# Autodesk Inventor assembly: Full Energy Chain Tensioner
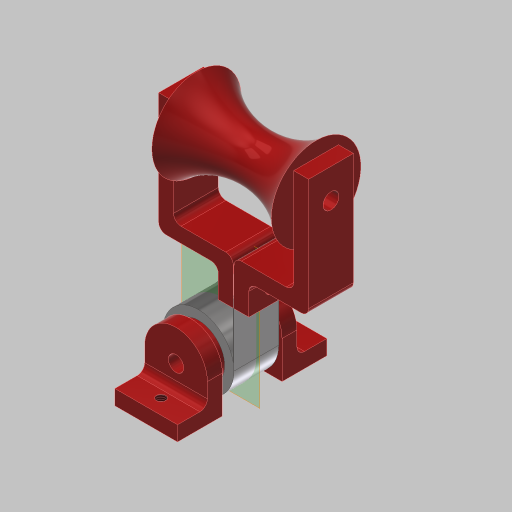
[picture p0: Inventor's stored thumbnail of the model, 512x512]
Saved by Autodesk Inventor 2023.5 (Build 275446000, 446)
## iProperties
Created: 2025-02-13
Part Number: Full Energy Chain Tensioner
Document SubType Name: Assembly
Designer: slick
Author: slick
## Documents named in this file (5)
- C:\Users\slick\OneDrive\Desktop\2025-ReefScape---CAD\Elevator\EL2\Full Energy Chain Tensioner.iam
- C:\Users\slick\OneDrive\Desktop\2025-ReefScape---CAD\Elevator\EL2\Energy Chain Tensioner piece.iam
- C:\Users\slick\OneDrive\Desktop\2025-ReefScape---CAD\Elevator\EL2\EL2-030.ipt
- C:\Users\slick\OneDrive\Desktop\2025-ReefScape---CAD\Elevator\EL2\EL2-029.ipt
- C:\Users\slick\OneDrive\Desktop\2025-ReefScape---CAD\COMMON PARTS\BEARINGS\Ball Bearing 1_4x11_16x5_16 Sealed 1602DC 1602-2RS.ipt
## Components (6 placed, 4 different names)
1. Energy Chain Tensioner piece:1 [sub-assembly] — Mate:1, Mate:2, Mate:3, Angle:1
2. EL2-030:1 — Flush:1, Flush:2, Mate:2, Angle:1, Mate:7
3. EL2-030:2 — Flush:1, Flush:2, Mate:1, Mate:3, Mate:6
4. EL2-029:1 — Mate:4, Mate:5, Flush:3, Flush:4
5. Ball Bearing 1_4x11_16x5_16 Sealed 1602DC 1602-2RS:1 — Mate:5, Flush:3, Mate:7
6. Ball Bearing 1_4x11_16x5_16 Sealed 1602DC 1602-2RS:2 — Mate:4, Flush:4, Mate:6
## Relationships (12: Mate 7, Flush 4, Angle 1)
- Flush:1: EL2-030:1 ↔ EL2-030:2
- Flush:2: EL2-030:1 ↔ EL2-030:2
- Mate:1: Energy Chain Tensioner piece:1 ↔ EL2-030:2
- Mate:2: Energy Chain Tensioner piece:1 ↔ EL2-030:1
- Mate:3: Energy Chain Tensioner piece:1 ↔ EL2-030:2
- Angle:1 (0 deg): Energy Chain Tensioner piece:1 ↔ EL2-030:1
- Mate:4: EL2-029:1 ↔ Ball Bearing 1_4x11_16x5_16 Sealed 1602DC 1602-2RS:2
- Mate:5: EL2-029:1 ↔ Ball Bearing 1_4x11_16x5_16 Sealed 1602DC 1602-2RS:1
- Flush:3: EL2-029:1 ↔ Ball Bearing 1_4x11_16x5_16 Sealed 1602DC 1602-2RS:1
- Flush:4: EL2-029:1 ↔ Ball Bearing 1_4x11_16x5_16 Sealed 1602DC 1602-2RS:2
- Mate:6: EL2-030:2 ↔ Ball Bearing 1_4x11_16x5_16 Sealed 1602DC 1602-2RS:2
- Mate:7: EL2-030:1 ↔ Ball Bearing 1_4x11_16x5_16 Sealed 1602DC 1602-2RS:1
